# Autodesk Inventor assembly: 28아이들러
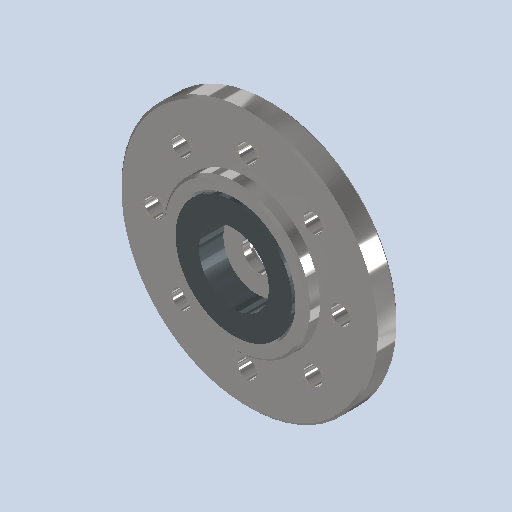
[picture p0: Inventor's stored thumbnail of the model, 512x512]
Saved by Autodesk Inventor 2024 (Build 280153000, 153)
## iProperties
Created: 2022-08-09
Part Number: 28아이들러
Document SubType Name: Assembly
Designer: 박지훈
Mass: 3 g
Surface Area: 13.0954 cm^2
Volume: 0.790597 cm^3
Density: 3.7946 g/cm^3
Author: 박지훈
## Documents named in this file (4)
- C:\Users\Eungang\Documents\Inventor\FIGHTING_ROBOT_FINAL\부품\아이들러\28아이들러.iam
- C:\Users\Eungang\Documents\Inventor\FIGHTING_ROBOT_FINAL\부품\아이들러\MF106ZZ.ipt
- C:\Users\Eungang\Documents\Inventor\FIGHTING_ROBOT_FINAL\부품\아이들러\RX28-CAP.ipt
- C:\Users\Eungang\Documents\Inventor\FIGHTING_ROBOT_FINAL\부품\아이들러\HN07-i101.ipt
## Components (3 placed, 3 different names)
1. MF106ZZ:1 — 삽입:2, 삽입:3
2. RX28-CAP:1 — 삽입:2
3. HN07-i101:1 — 삽입:3
## Relationships (2: Insert 2)
- 삽입:2 [Insert]: MF106ZZ:1 ↔ RX28-CAP:1
- 삽입:3 [Insert]: MF106ZZ:1 ↔ HN07-i101:1
